# Autodesk Inventor assembly: Cube 1x1 V5 (Mirror Vertical)
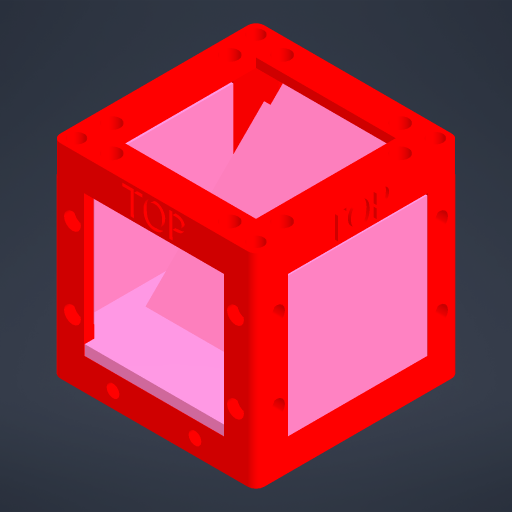
[picture p0: Inventor's stored thumbnail of the model, 512x512]
Saved by Autodesk Inventor 2023.4 (Build 274418000, 418)
## iProperties
Created: 2022-08-13
Part Number: Cube 1x1 V5 (Mirror Vertical)
Document SubType Name: Assembly
Designer: xSibe
Author: xSibe
## Documents named in this file (4)
- C:\.Laptop\.Work\Projects\Project Protocube\1 Autodesk\1 Cubes\Mirror\Cube 1x1 V5 (Mirror Vertical).iam
- C:\.Laptop\.Work\Projects\Project Protocube\1 Autodesk\1 Cubes\Mirror\Mirror Base Vertical.ipt
- C:\.Laptop\.Work\Projects\Project Protocube\1 Autodesk\1 Cubes\Mirror\Mirror Plate Vertical.ipt
- C:\.Laptop\.Work\Projects\Project Protocube\1 Autodesk\1 Cubes\Cubes\Cube 1x1 V5.iam
## Components (3 placed, 3 different names)
1. Mirror Base Vertical:1 — Mate:4, Mate:5, Flush:1
2. Mirror Plate Vertical:1 — Mate:6, Flush:2, Mate:7
3. Cube 1x1 V5:1 [sub-assembly]
## Relationships (6: Mate 4, Flush 2)
- Mate:4: Mirror Base Vertical:1
- Mate:5: Mirror Base Vertical:1
- Flush:1: Mirror Base Vertical:1
- Mate:6: Mirror Plate Vertical:1
- Flush:2: Mirror Plate Vertical:1
- Mate:7: Mirror Plate Vertical:1
